# Autodesk Inventor assembly: CollectorPrototype
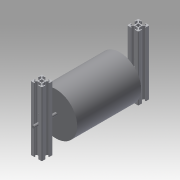
[picture p0: Inventor's stored thumbnail of the model, 180x180]
Saved by Autodesk Inventor 2016 (Build 200138000, 138)
## iProperties
Created: 2016-12-07
Part Number: CollectorPrototype
Document SubType Name: Assembly
Designer: Delta
Author: Delta
## Documents named in this file (5)
- C:\Robotics\CAD\2016-17_CAD\CollectorPrototype.iam
- C:\Robotics\CAD\COTSParts\Bosch Extrusion\Bosch 20x20 - 4.5 Part.Shoot.ipt
- C:\Robotics\CAD\2016-17_CAD\6InchAx.ipt
- C:\Robotics\CAD\2016-17_CAD\CollectorBrush.ipt
- C:\Robotics\CAD\COTSParts\Tetrix\Tetrix Gear 40T.ipt
## Components (5 placed, 4 different names)
1. Bosch 20x20 - 4.5 Part.Shoot:1 — Mate:1, Flush:1, Flush:2, Insert:1
2. Bosch 20x20 - 4.5 Part.Shoot:2 — Mate:1, Flush:1, Flush:2
3. 6InchAx:1 — Insert:1, Insert:2, Mate:3
4. CollectorBrush:1 — Insert:2, Mate:2
5. Tetrix Gear 40T:1 — Mate:2, Mate:3
## Relationships (7: Mate 3, Flush 2, Insert 2)
- Mate:1 (152.4 mm): Bosch 20x20 - 4.5 Part.Shoot:1 ↔ Bosch 20x20 - 4.5 Part.Shoot:2
- Flush:1: Bosch 20x20 - 4.5 Part.Shoot:1 ↔ Bosch 20x20 - 4.5 Part.Shoot:2
- Flush:2: Bosch 20x20 - 4.5 Part.Shoot:1 ↔ Bosch 20x20 - 4.5 Part.Shoot:2
- Insert:1 (-10.8966 mm): Bosch 20x20 - 4.5 Part.Shoot:1 ↔ 6InchAx:1
- Insert:2 (48.26 mm): 6InchAx:1 ↔ CollectorBrush:1
- Mate:2: CollectorBrush:1 ↔ Tetrix Gear 40T:1
- Mate:3: 6InchAx:1 ↔ Tetrix Gear 40T:1
